# Autodesk Inventor assembly: BBM Staging Plate Assembly
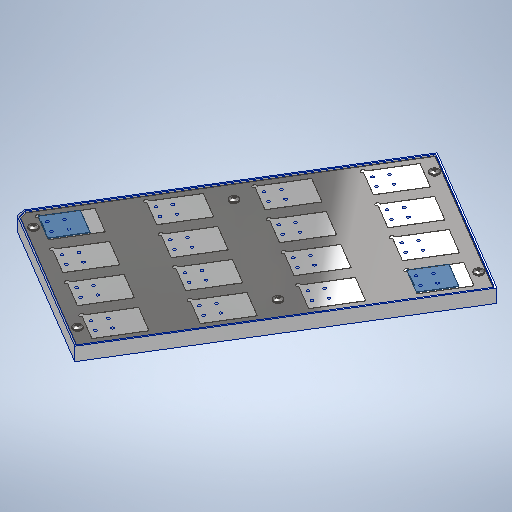
[picture p0: Inventor's stored thumbnail of the model, 512x512]
Saved by Autodesk Inventor 2025 (Build 290162000, 162)
## iProperties
Created: 2021-01-11
Part Number: BBM Staging Plate Assembly
Document SubType Name: Assembly
Designer: caleb
Author: caleb
## Documents named in this file (5)
- C:\Users\cfang\Desktop\nebraska-silicon-lab\Hardware\ETL\Module Assembly\BBM Staging Plate - V2\BBM Staging Plate Assembly - V2.iam
- C:\Users\cfang\Desktop\nebraska-silicon-lab\Hardware\ETL\Module Assembly\BBM Staging Plate - V2\BBM Staging Plate - V2.ipt
- C:\Users\cfang\Desktop\nebraska-silicon-lab\Hardware\ETL\Module Assembly\BBM Staging Plate - V2\BBM Staging Plate Stencil - V2.ipt
- C:\Users\cfang\Desktop\nebraska-silicon-lab\Hardware\ETL\Module Assembly\BBM Staging Plate - V2\F10112319--_1-MODULE_ CMS2 ETL_ PIXEL SENSOR READOUT CHIP.ipt
- C:\Users\cfang\Desktop\nebraska-silicon-lab\Hardware\ETL\Module Assembly\BBM Staging Plate - V2\90116A151_316 Stainless Steel Pan Head Phillips Screws\90116A151_316 Stainless Steel Pan Head Phillips Screws.ipt
## Components (10 placed, 4 different names)
1. BBM Staging Plate - V2:1 — Mate:11, Mate:12, Mate:13, Mate:14, Mate:15
2. BBM Staging Plate Stencil - V2:1 — Mate:6, Mate:7, Mate:9, Mate:10, Mate:11, Mate:12, Mate:13, Insert:1, Insert:2, Insert:3, Insert:4, Insert:5, Insert:6
3. F10112319--_1-MODULE_ CMS2 ETL_ PIXEL SENSOR READOUT CHIP:1 — Mate:6, Mate:7, Mate:15
4. F10112319--_1-MODULE_ CMS2 ETL_ PIXEL SENSOR READOUT CHIP:2 — Mate:9, Mate:10, Mate:14
5. 90116A151_316 Stainless Steel Pan Head Phillips Screws:1 — Insert:1
6. 90116A151_316 Stainless Steel Pan Head Phillips Screws:2 — Insert:2
7. 90116A151_316 Stainless Steel Pan Head Phillips Screws:3 — Insert:3
8. 90116A151_316 Stainless Steel Pan Head Phillips Screws:4 — Insert:4
9. 90116A151_316 Stainless Steel Pan Head Phillips Screws:5 — Insert:6
10. 90116A151_316 Stainless Steel Pan Head Phillips Screws:6 — Insert:5
## Relationships (15: Mate 9, Insert 6)
- Mate:6: BBM Staging Plate Stencil - V2:1 ↔ F10112319--_1-MODULE_ CMS2 ETL_ PIXEL SENSOR READOUT CHIP:1
- Mate:7: BBM Staging Plate Stencil - V2:1 ↔ F10112319--_1-MODULE_ CMS2 ETL_ PIXEL SENSOR READOUT CHIP:1
- Mate:9: BBM Staging Plate Stencil - V2:1 ↔ F10112319--_1-MODULE_ CMS2 ETL_ PIXEL SENSOR READOUT CHIP:2
- Mate:10: BBM Staging Plate Stencil - V2:1 ↔ F10112319--_1-MODULE_ CMS2 ETL_ PIXEL SENSOR READOUT CHIP:2
- Mate:11: BBM Staging Plate - V2:1 ↔ BBM Staging Plate Stencil - V2:1
- Mate:12 (0.5 mm): BBM Staging Plate - V2:1 ↔ BBM Staging Plate Stencil - V2:1
- Mate:13 (0.5 mm): BBM Staging Plate - V2:1 ↔ BBM Staging Plate Stencil - V2:1
- Mate:14: BBM Staging Plate - V2:1 ↔ F10112319--_1-MODULE_ CMS2 ETL_ PIXEL SENSOR READOUT CHIP:2
- Mate:15: BBM Staging Plate - V2:1 ↔ F10112319--_1-MODULE_ CMS2 ETL_ PIXEL SENSOR READOUT CHIP:1
- Insert:1: BBM Staging Plate Stencil - V2:1 ↔ 90116A151_316 Stainless Steel Pan Head Phillips Screws:1
- Insert:2: BBM Staging Plate Stencil - V2:1 ↔ 90116A151_316 Stainless Steel Pan Head Phillips Screws:2
- Insert:3: BBM Staging Plate Stencil - V2:1 ↔ 90116A151_316 Stainless Steel Pan Head Phillips Screws:3
- Insert:4: BBM Staging Plate Stencil - V2:1 ↔ 90116A151_316 Stainless Steel Pan Head Phillips Screws:4
- Insert:5: BBM Staging Plate Stencil - V2:1 ↔ 90116A151_316 Stainless Steel Pan Head Phillips Screws:6
- Insert:6: BBM Staging Plate Stencil - V2:1 ↔ 90116A151_316 Stainless Steel Pan Head Phillips Screws:5
